# Autodesk Inventor assembly: Motor Mount with Motor
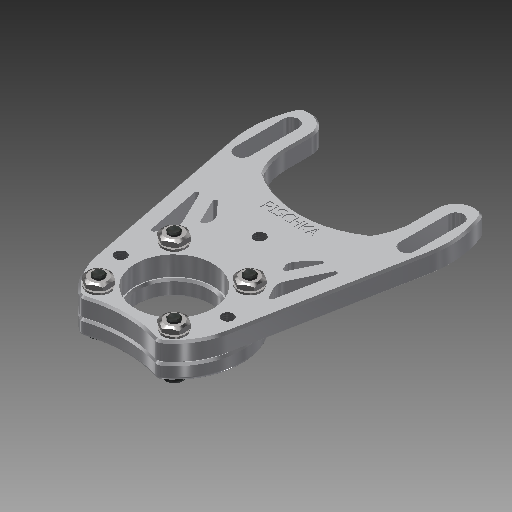
[picture p0: Inventor's stored thumbnail of the model, 512x512]
Saved by Autodesk Inventor 2019.3 (Build 233278000, 278)
## iProperties
Created: 2019-03-01
Part Number: Motor Mount with Motor
Document SubType Name: Assembly
Designer: Petar
Mass: 37.7633 g
Surface Area: 102.459 cm^2
Volume: 12.7696 cm^3
Density: 2.95729 g/cm^3
Author: Petar
## Documents named in this file (7)
- D:\OMG\E-Board\CAD\Inventor\Motor Mount - 225.iam
- D:\OMG\E-Board\CAD\Inventor\Mechanical Components\Motor Mount.ipt
- D:\OMG\E-Board\CAD\Inventor\Motor Mount\Design Accelerator\Bolted Connection1.iam
- D:\OMG\E-Board\CAD\Inventor\Motor Mount\Design Accelerator\Bolted Connection2.iam
- D:\OMG\E-Board\CAD\Inventor\Motor Mount\Design Accelerator\Bolted Connection3.iam
- D:\OMG\E-Board\CAD\Inventor\Motor Mount\Design Accelerator\Bolted Connection4.iam
- D:\OMG\E-Board\CAD\Inventor\Mechanical Components\Motor Holder v3 - 225.ipt
## Components (6 placed, 3 different names)
1. Motor Holder v3 - 225:1 — Mate:4, Mate:5, Mate:6, Mate:8, Mate:10, Mate:12, Mate:14
2. Motor Mount:1 — Mate:4, Mate:5, Mate:6, Mate:7, Mate:9, Mate:11, Mate:13
3. Bolted Connection:1 [sub-assembly] — Mate:7, Mate:8
4. Bolted Connection:2 [sub-assembly] — Mate:9, Mate:10
5. Bolted Connection:3 [sub-assembly] — Mate:11, Mate:12
6. Bolted Connection:4 [sub-assembly] — Mate:13, Mate:14
## Relationships (11: Mate 11)
- Mate:4: Motor Holder v3 - 225:1 ↔ Motor Mount:1
- Mate:5: Motor Holder v3 - 225:1 ↔ Motor Mount:1
- Mate:6: Motor Holder v3 - 225:1 ↔ Motor Mount:1
- Mate:7: Motor Mount:1 ↔ Bolted Connection:1
- Mate:8: Motor Holder v3 - 225:1 ↔ Bolted Connection:1
- Mate:9: Motor Mount:1 ↔ Bolted Connection:2
- Mate:10: Motor Holder v3 - 225:1 ↔ Bolted Connection:2
- Mate:11: Motor Mount:1 ↔ Bolted Connection:3
- Mate:12: Motor Holder v3 - 225:1 ↔ Bolted Connection:3
- Mate:13: Motor Mount:1 ↔ Bolted Connection:4
- Mate:14: Motor Holder v3 - 225:1 ↔ Bolted Connection:4
